# Autodesk Inventor assembly: Final_Assembly
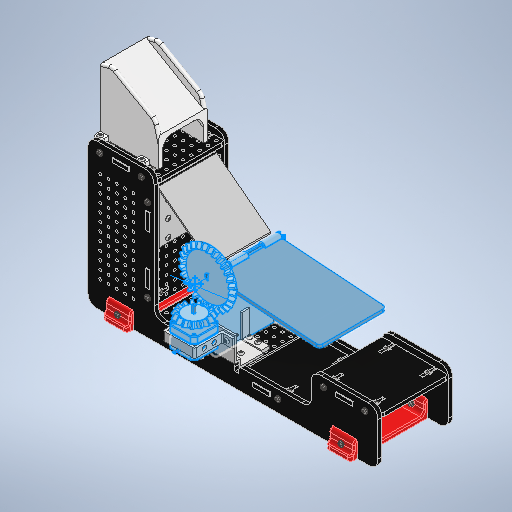
[picture p0: Inventor's stored thumbnail of the model, 512x512]
Saved by Autodesk Inventor 2025.1 (Build 291241000, 241)
## iProperties
Created: 2024-10-22
Part Number: Final_Assembly
Document SubType Name: Assembly
Designer: vedan
Author: vedan
## Documents named in this file (11)
- C:\Users\hanna\OneDrive - McMaster University\Documents\ENG 1P13A\Project 1\Final_Assembly.iam
- C:\Users\hanna\OneDrive - McMaster University\Documents\ENG 1P13A\Project 1\New folder (1)\Mechanism Platform.iam
- C:\Users\hanna\OneDrive - McMaster University\Documents\ENG 1P13A\Project 1\New folder (1)\mechanism.ipt
- C:\Users\hanna\OneDrive - McMaster University\Documents\ENG 1P13A\Project 1\New folder (1)\Hinge Assembly.iam
- C:\Users\hanna\OneDrive - McMaster University\Documents\ENG 1P13A\Project 1\Autodesk Inventor CAD Part Models\Mounting Hardware\Rotary Actuator Mount.ipt
- C:\Users\hanna\OneDrive - McMaster University\Documents\ENG 1P13A\Project 1\Autodesk Inventor CAD Part Models\Fasteners\2. Plate Fasteners\2. Plate Fasteners\M4 x 16mm Machine Screw.ipt
- C:\Users\hanna\OneDrive - McMaster University\Documents\ENG 1P13A\Project 1\P1D1_2Ramp.ipt
- C:\Users\hanna\OneDrive - McMaster University\Documents\ENG 1P13A\Project 1\RotaryActBracket.ipt
- C:\Users\hanna\OneDrive - McMaster University\Documents\ENG 1P13A\Project 1\New folder (1)\M4 x 20mm Machine Screw.ipt
- C:\Users\hanna\OneDrive - McMaster University\Documents\ENG 1P13A\Project 1\Support.ipt
- C:\Users\hanna\OneDrive - McMaster University\Documents\ENG 1P13A\Project 1\Autodesk Inventor CAD Part Models\Fasteners\2. Plate Fasteners\2. Plate Fasteners\M4 Nut.ipt
## Components (50 placed, 10 different names)
1. mechanism:1 — Angle:16, Mate:1, Mate:2, Angle:17
2. Mechanism Platform:1 [sub-assembly] — Flush:1, Flush:2, Flush:7, Angle:16, Mate:1, Mate:2, Mate:3, Mate:4, Mate:24, Mate:25, Mate:29, Mate:33, Mate:34, Mate:35, Mate:38, Mate:41, Mate:42, Mate:43, Mate:44, Insert:21, Insert:22, Insert:23, Insert:24, Insert:25, Insert:26, Insert:27, Insert:28, Insert:29, Insert:30, Insert:31, Insert:32, Insert:33, Insert:34, Insert:35, Insert:36, Insert:37, Insert:40, Insert:41, Mate:47, Mate:48, Mate:49, Mate:51, Mate:52, Mate:53, Insert:42, Angle:18
3. Hinge Assembly:1 [sub-assembly] — Mate:3, Mate:4, Angle:17, Mate:6, Mate:7, Mate:12, Mate:32, Mate:50, Angle:18
4. Rotary Actuator Mount:1 — Mate:6, Mate:7, Mate:12, Insert:7, Insert:18
5. M4 x 16mm Machine Screw:1 — Mate:28, Insert:7
6. P1D1_2Ramp:1 — Mate:24, Insert:1, Insert:2, Insert:3, Insert:4, Insert:5, Insert:6, Mate:47
7. RotaryActBracket:1 — Mate:25, Mate:28, Mate:29, Insert:19, Insert:20, Insert:38, Insert:39
8. M4 x 20mm Machine Screw:1 — Insert:1
9. M4 x 20mm Machine Screw:2 — Insert:2
10. M4 x 20mm Machine Screw:3 — Insert:3
11. M4 x 20mm Machine Screw:4 — Insert:5, Mate:48
12. M4 x 20mm Machine Screw:5 — Insert:4
13. M4 x 20mm Machine Screw:6 — Insert:6, Mate:49
14. Support:2 — Mate:33, Mate:34, Mate:35, Insert:10, Insert:17
15. Support:3 — Mate:32, Mate:38, Mate:41, Mate:42, Insert:11, Insert:12
16. Support:4 — Mate:43, Insert:15, Insert:16, Mate:50, Mate:51
17. Support:5 — Mate:44, Insert:13, Insert:14, Mate:52
18. M4 x 16mm Machine Screw:2 — Insert:14, Mate:53
19. M4 x 16mm Machine Screw:3 — Insert:11
20. M4 x 16mm Machine Screw:4 — Insert:13
21. M4 x 16mm Machine Screw:5 — Insert:17
22. M4 x 16mm Machine Screw:6 — Insert:10
23. M4 x 16mm Machine Screw:7 — Insert:15
24. M4 x 16mm Machine Screw:8 — Insert:12
25. M4 x 16mm Machine Screw:9 — Insert:16
26. M4 Nut:1 — Insert:33
27. M4 Nut:2 — Insert:30
28. M4 Nut:3 — Insert:27
29. M4 Nut:4 — Insert:28
30. M4 Nut:5 — Insert:25
31. M4 Nut:6 — Insert:24
32. M4 Nut:7 — Insert:26
33. M4 Nut:8 — Insert:31
34. M4 Nut:9 — Insert:19
35. M4 Nut:10 — Insert:21
36. M4 Nut:11 — Insert:42
37. M4 Nut:12 — Insert:32
38. M4 Nut:13 — Insert:22
39. M4 Nut:14 — Insert:20
40. M4 Nut:15 — Insert:23
41. M4 Nut:16 — Insert:29
42. M4 x 16mm Machine Screw:10 — Insert:39
43. M4 x 16mm Machine Screw:11 — Insert:38
44. M4 x 16mm Machine Screw:12 — Insert:18
45. M4 Nut:17 — Insert:35
46. M4 Nut:18 — Insert:34
47. M4 Nut:19 — Insert:36
48. M4 Nut:20 — Insert:37
49. M4 Nut:21 — Insert:41
50. M4 Nut:22 — Insert:40
## Relationships (73: Insert 40, Mate 27, Flush 3, Angle 3)
- Flush:1: Mechanism Platform:1
- Flush:2: Mechanism Platform:1
- Flush:7: Mechanism Platform:1
- Angle:16 (180 deg): mechanism:1 ↔ Mechanism Platform:1
- Mate:1: mechanism:1 ↔ Mechanism Platform:1
- Mate:2: mechanism:1 ↔ Mechanism Platform:1
- Mate:3: Mechanism Platform:1 ↔ Hinge Assembly:1
- Mate:4: Mechanism Platform:1 ↔ Hinge Assembly:1
- Angle:17 (180 deg): mechanism:1 ↔ Hinge Assembly:1
- Mate:6: Hinge Assembly:1 ↔ Rotary Actuator Mount:1
- Mate:7: Hinge Assembly:1 ↔ Rotary Actuator Mount:1
- Mate:12: Hinge Assembly:1 ↔ Rotary Actuator Mount:1
- Mate:24: Mechanism Platform:1 ↔ P1D1_2Ramp:1
- Mate:25: Mechanism Platform:1 ↔ RotaryActBracket:1
- Insert:1: P1D1_2Ramp:1 ↔ M4 x 20mm Machine Screw:1
- Insert:2: P1D1_2Ramp:1 ↔ M4 x 20mm Machine Screw:2
- Insert:3: P1D1_2Ramp:1 ↔ M4 x 20mm Machine Screw:3
- Insert:4: P1D1_2Ramp:1 ↔ M4 x 20mm Machine Screw:5
- Insert:5: P1D1_2Ramp:1 ↔ M4 x 20mm Machine Screw:4
- Insert:6: P1D1_2Ramp:1 ↔ M4 x 20mm Machine Screw:6
- Mate:28: M4 x 16mm Machine Screw:1 ↔ RotaryActBracket:1
- Mate:29: Mechanism Platform:1 ↔ RotaryActBracket:1
- Insert:7: Rotary Actuator Mount:1 ↔ M4 x 16mm Machine Screw:1
- Mate:32: Hinge Assembly:1 ↔ Support:3
- Mate:33: Mechanism Platform:1 ↔ Support:2
- Mate:34: Mechanism Platform:1 ↔ Support:2
- Mate:35: Mechanism Platform:1 ↔ Support:2
- Mate:38: Mechanism Platform:1 ↔ Support:3
- Insert:10: Support:2 ↔ M4 x 16mm Machine Screw:6
- Mate:41: Mechanism Platform:1 ↔ Support:3
- Mate:42: Mechanism Platform:1 ↔ Support:3
- Insert:11: Support:3 ↔ M4 x 16mm Machine Screw:3
- Insert:12: Support:3 ↔ M4 x 16mm Machine Screw:8
- Mate:43: Mechanism Platform:1 ↔ Support:4
- Mate:44: Mechanism Platform:1 ↔ Support:5
- Insert:13: Support:5 ↔ M4 x 16mm Machine Screw:4
- Insert:14: Support:5 ↔ M4 x 16mm Machine Screw:2
- Insert:15: Support:4 ↔ M4 x 16mm Machine Screw:7
- Insert:16: Support:4 ↔ M4 x 16mm Machine Screw:9
- Insert:17: Support:2 ↔ M4 x 16mm Machine Screw:5
- Insert:18: Rotary Actuator Mount:1 ↔ M4 x 16mm Machine Screw:12
- Insert:19: RotaryActBracket:1 ↔ M4 Nut:9
- Insert:20: RotaryActBracket:1 ↔ M4 Nut:14
- Insert:21: Mechanism Platform:1 ↔ M4 Nut:10
- Insert:22: Mechanism Platform:1 ↔ M4 Nut:13
- Insert:23: Mechanism Platform:1 ↔ M4 Nut:15
- Insert:24: Mechanism Platform:1 ↔ M4 Nut:6
- Insert:25: Mechanism Platform:1 ↔ M4 Nut:5
- Insert:26: Mechanism Platform:1 ↔ M4 Nut:7
- Insert:27: Mechanism Platform:1 ↔ M4 Nut:3
- Insert:28: Mechanism Platform:1 ↔ M4 Nut:4
- Insert:29: Mechanism Platform:1 ↔ M4 Nut:16
- Insert:30: Mechanism Platform:1 ↔ M4 Nut:2
- Insert:31: Mechanism Platform:1 ↔ M4 Nut:8
- Insert:32: Mechanism Platform:1 ↔ M4 Nut:12
- Insert:33: Mechanism Platform:1 ↔ M4 Nut:1
- Insert:34: Mechanism Platform:1 ↔ M4 Nut:18
- Insert:35: Mechanism Platform:1 ↔ M4 Nut:17
- Insert:36: Mechanism Platform:1 ↔ M4 Nut:19
- Insert:37: Mechanism Platform:1 ↔ M4 Nut:20
- Insert:38: RotaryActBracket:1 ↔ M4 x 16mm Machine Screw:11
- Insert:39: RotaryActBracket:1 ↔ M4 x 16mm Machine Screw:10
- Insert:40: Mechanism Platform:1 ↔ M4 Nut:22
- Insert:41: Mechanism Platform:1 ↔ M4 Nut:21
- Mate:47: Mechanism Platform:1 ↔ P1D1_2Ramp:1
- Mate:48: Mechanism Platform:1 ↔ M4 x 20mm Machine Screw:4
- Mate:49: Mechanism Platform:1 ↔ M4 x 20mm Machine Screw:6
- Mate:50: Hinge Assembly:1 ↔ Support:4
- Mate:51: Mechanism Platform:1 ↔ Support:4
- Mate:52: Mechanism Platform:1 ↔ Support:5
- Mate:53: Mechanism Platform:1 ↔ M4 x 16mm Machine Screw:2
- Insert:42: Mechanism Platform:1 ↔ M4 Nut:11
- Angle:18 (0 deg): Mechanism Platform:1 ↔ Hinge Assembly:1
